# Autodesk Inventor assembly: Mech Motor_Wheel
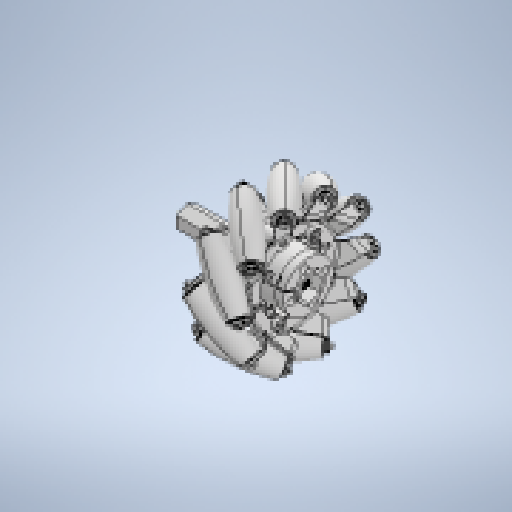
[picture p0: Inventor's stored thumbnail of the model, 512x512]
Saved by Autodesk Inventor 2023 (Build 270158000, 158)
## iProperties
Created: 2021-10-04
Part Number: Mech Motor_Wheel
Document SubType Name: Assembly
Designer: TakeHomePC
Author: TakeHomePC
## Documents named in this file (7)
- C:\Users\matt\Documents\Inventor\FTC\2022-23 FTC\Mech Chassis\Mech Motor_Wheel.iam
- C:\Users\matt\Documents\Inventor\FTC\2022-23 FTC\500H x 50mm.ipt
- C:\Users\matt\Documents\Inventor\FTC\2022-23 FTC\Mech Chassis\GoBilda Mec Wheel\3213-3606-0002\3606-0000-0096 assembly.iam
- C:\Users\matt\Documents\Inventor\FTC\2022-23 FTC\Mech Chassis\GoBilda Mech Hub 0500 Hex.ipt
- C:\Users\matt\Documents\Inventor\FTC\2022-23 FTC\Fasteners\M6 x 10.ipt
- C:\Users\matt\Documents\Inventor\FTC\2022-23 FTC\Fasteners\M5 x 25.ipt
- C:\Users\matt\Documents\Inventor\FTC\2022-23 FTC\Mech Chassis\GoBilda Mech Hub 0500 Hex Spacer  inserts.ipt
## Components (9 placed, 6 different names)
1. 500H x 50mm:2 — Mate:1, Mate:3, Mate:5, Mate:6, Angle:1
2. 3606-0000-0096 assembly:1 [sub-assembly] — Mate:1, Mate:2, Mate:4, Mate:7
3. GoBilda Mech Hub 0500 Hex Spacer  inserts:1 — Mate:2, Mate:3, Mate:4, Mate:8, Angle:1
4. GoBilda Mech Hub 0500 Hex:1 — Mate:5, Mate:6, Mate:7, Mate:8, Mate:9, Mate:10, Mate:11, Mate:12, Mate:13, Mate:14, Mate:15, Mate:16, Mate:17, Mate:18
5. M6 x 10:1 — Mate:9, Mate:10
6. M5 x 25:1 — Mate:11, Mate:12
7. M5 x 25:2 — Mate:15, Mate:16
8. M5 x 25:3 — Mate:14, Mate:17
9. M5 x 25:4 — Mate:13, Mate:18
## Relationships (19: Mate 18, Angle 1)
- Mate:1: 500H x 50mm:2 ↔ 3606-0000-0096 assembly:1
- Mate:2: 3606-0000-0096 assembly:1 ↔ GoBilda Mech Hub 0500 Hex Spacer  inserts:1
- Mate:3: 500H x 50mm:2 ↔ GoBilda Mech Hub 0500 Hex Spacer  inserts:1
- Mate:4: 3606-0000-0096 assembly:1 ↔ GoBilda Mech Hub 0500 Hex Spacer  inserts:1
- Mate:5: 500H x 50mm:2 ↔ GoBilda Mech Hub 0500 Hex:1
- Mate:6: 500H x 50mm:2 ↔ GoBilda Mech Hub 0500 Hex:1
- Mate:7: 3606-0000-0096 assembly:1 ↔ GoBilda Mech Hub 0500 Hex:1
- Mate:8: GoBilda Mech Hub 0500 Hex Spacer  inserts:1 ↔ GoBilda Mech Hub 0500 Hex:1
- Angle:1 (0 deg): 500H x 50mm:2 ↔ GoBilda Mech Hub 0500 Hex Spacer  inserts:1
- Mate:9: GoBilda Mech Hub 0500 Hex:1 ↔ M6 x 10:1
- Mate:10: GoBilda Mech Hub 0500 Hex:1 ↔ M6 x 10:1
- Mate:11: GoBilda Mech Hub 0500 Hex:1 ↔ M5 x 25:1
- Mate:12: GoBilda Mech Hub 0500 Hex:1 ↔ M5 x 25:1
- Mate:13: GoBilda Mech Hub 0500 Hex:1 ↔ M5 x 25:4
- Mate:14: GoBilda Mech Hub 0500 Hex:1 ↔ M5 x 25:3
- Mate:15: GoBilda Mech Hub 0500 Hex:1 ↔ M5 x 25:2
- Mate:16: GoBilda Mech Hub 0500 Hex:1 ↔ M5 x 25:2
- Mate:17: GoBilda Mech Hub 0500 Hex:1 ↔ M5 x 25:3
- Mate:18: GoBilda Mech Hub 0500 Hex:1 ↔ M5 x 25:4
